# Autodesk Inventor assembly: 組合1
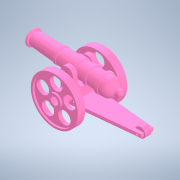
[picture p0: Inventor's stored thumbnail of the model, 180x180]
Saved by Autodesk Inventor 2022 (Build 260153000, 153)
## iProperties
Created: 2023-05-26
Part Number: 組合1
Document SubType Name: Assembly
Designer: USER
Author: USER
## Documents named in this file (9)
- C:\Users\USER\Desktop\cannon-cad\cannon_combine.iam
- C:\Users\USER\Desktop\cannon-cad\4.holder.ipt
- C:\Users\USER\Desktop\cannon-cad\7.barbette.ipt
- C:\Users\USER\Desktop\cannon-cad\8.wheel.ipt
- C:\Users\USER\Desktop\cannon-cad\1.barrel.ipt
- C:\Users\USER\Desktop\cannon-cad\3.breech.ipt
- C:\Users\USER\Desktop\cannon-cad\9.tail_wheel.ipt
- C:\Users\USER\Desktop\cannon-cad\2.bolt.ipt
- C:\Users\USER\Desktop\cannon-cad\6.ring.ipt
## Components (10 placed, 8 different names)
1. 4.holder:1 — 貼合:1, 貼合:2, 貼合:3, 貼合:17, 貼合:18, 貼合:19, 貼合:20, 貼合:21
2. 7.barbette:1 — 貼合:1, 貼合:2, 貼合:3, 貼合:8, 貼合:9, 貼合:10, 貼合:22, 貼合:23, 貼合:24, 貼合:25
3. 1. 砲管:1 — 貼合:8, 貼合:9, 貼合:10, 貼合:11, 貼合:12
4. 3.breech:1 — 貼合:11, 貼合:12
5. 9.tail_wheel:1 — 貼合:17, 貼合:18, 貼合:19
6. 2. 螺栓:1 — 貼合:20, 貼合:21
7. 6.ring:1 — 貼合:22, 貼合:23, 貼合:26, 貼合:27
8. 6.ring:2 — 貼合:24, 貼合:25, 貼合:28, 貼合:29
9. 8.wheel:1 — 貼合:26, 貼合:27
10. 8.wheel:2 — 貼合:28, 貼合:29
## Relationships (21: Mate 21)
- 貼合:1 [Mate]: 4.holder:1 ↔ 7.barbette:1
- 貼合:2 [Mate]: 4.holder:1 ↔ 7.barbette:1
- 貼合:3 [Mate]: 4.holder:1 ↔ 7.barbette:1
- 貼合:8 [Mate]: 7.barbette:1 ↔ 1. 砲管:1
- 貼合:9 [Mate]: 7.barbette:1 ↔ 1. 砲管:1
- 貼合:10 [Mate]: 7.barbette:1 ↔ 1. 砲管:1
- 貼合:11 [Mate]: 1. 砲管:1 ↔ 3.breech:1
- 貼合:12 [Mate]: 1. 砲管:1 ↔ 3.breech:1
- 貼合:17 [Mate]: 4.holder:1 ↔ 9.tail_wheel:1
- 貼合:18 [Mate]: 4.holder:1 ↔ 9.tail_wheel:1
- 貼合:19 [Mate]: 4.holder:1 ↔ 9.tail_wheel:1
- 貼合:20 [Mate]: 4.holder:1 ↔ 2. 螺栓:1
- 貼合:21 [Mate]: 4.holder:1 ↔ 2. 螺栓:1
- 貼合:22 [Mate]: 7.barbette:1 ↔ 6.ring:1
- 貼合:23 [Mate]: 7.barbette:1 ↔ 6.ring:1
- 貼合:24 [Mate]: 7.barbette:1 ↔ 6.ring:2
- 貼合:25 [Mate]: 7.barbette:1 ↔ 6.ring:2
- 貼合:26 [Mate]: 6.ring:1 ↔ 8.wheel:1
- 貼合:27 [Mate]: 6.ring:1 ↔ 8.wheel:1
- 貼合:28 [Mate]: 6.ring:2 ↔ 8.wheel:2
- 貼合:29 [Mate]: 6.ring:2 ↔ 8.wheel:2
